# Autodesk Inventor assembly: robot
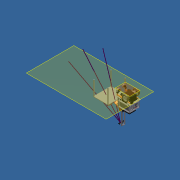
[picture p0: Inventor's stored thumbnail of the model, 180x180]
Saved by Autodesk Inventor 2012 (Build 160160000, 160)
## iProperties
Created: 2012-03-08
Part Number: robot
Document SubType Name: Assembly
Designer: esv
Mass: 187059 g
Surface Area: 125343 cm^2
Volume: 160092 cm^3
Density: 1.16845 g/cm^3
Author: esv
## Documents named in this file (22)
- C:\Users\Ed\Documents\masters\CAD\robot.iam
- C:\Users\Ed\Documents\masters\CAD\Frame\frame bracket.ipt
- C:\Users\Ed\Documents\masters\CAD\Invacare\invacare assy.iam
- C:\Users\Ed\Documents\masters\CAD\IRC5\IRC5_Compact.ipt
- C:\Users\Ed\Documents\masters\CAD\PC\PC.ipt
- C:\Users\Ed\Documents\masters\CAD\SICK\SICK LMS291.ipt
- C:\Users\Ed\Documents\masters\CAD\IRB120\IRB120.iam
- C:\Users\Ed\Documents\masters\CAD\Frame\back frame plate.ipt
- C:\Users\Ed\Documents\masters\CAD\Frame\front frame plate.ipt
- C:\Users\Ed\Documents\masters\CAD\Frame\top plate.ipt
- C:\Users\Ed\Documents\masters\CAD\Pneumatics\compressor\compressor.iam
- C:\Users\Ed\Documents\masters\CAD\Spike\Spike H.iam
- C:\Users\Ed\Documents\masters\CAD\Breaker\Breaker.iam
- C:\Users\Ed\Documents\masters\CAD\Router\router keepout.ipt
- C:\Users\Ed\Documents\masters\CAD\Frame\short frame bracket.ipt
- C:\Users\Ed\Documents\masters\CAD\base plate.iam
- C:\Users\Ed\Documents\masters\CAD\Gripper\gripper.iam
- C:\Users\Ed\Documents\masters\CAD\al_frame.iam
- C:\Users\Ed\Documents\masters\CAD\Gripper\gripper jaw.iam
- C:\Users\Ed\Documents\masters\CAD\Kinect\acrylic kinect bracket.iam
- C:\Users\Ed\Documents\masters\CAD\Kinect\Kinect.ipt
- C:\Users\Ed\Documents\masters\CAD\objects\table.ipt
## Components (26 placed, 21 different names)
1. frame bracket:1 — Flush:5, Mate:72, Flush:56, Mate:74, Mate:132
2. frame bracket:4 — Flush:5, Flush:57, Mate:75, Mate:76
3. invacare assy:1 [sub-assembly] — Flush:96, Tangent:8, Mate:97, Mate:143, Mate:144, Mate:145
4. IRC5_Compact:1 — Flush:2, Mate:122, Mate:126
5. PC:1 — Mate:36, Flush:63, Flush:91
6. SICK LMS291:1 — Mate:118, Insert:12
7. IRB120:1 [sub-assembly] — Insert:10, Insert:11, Mate:120, Tangent:7, Flush:145
8. back frame plate:1 — Flush:82, Insert:7, Flush:88, Flush:89, Flush:96, Tangent:8, Flush:98
9. back frame plate:2 — Insert:6, Flush:87, Flush:88, Flush:90, Flush:100
10. front frame plate:1 — Flush:57, Mate:75, Mate:76, Flush:89, Mate:97, Flush:98, Flush:99
11. front frame plate:2 — Mate:72, Flush:56, Mate:74, Flush:90, Flush:99, Flush:100
12. top plate:1 — Mate:36, Mate:80, Flush:63, Mate:81, Insert:1, Insert:2, Insert:3, Mate:82, Insert:4, Insert:5, Flush:64, Mate:121, Flush:85, Flush:86, Flush:91
13. compressor:1 [sub-assembly] — Mate:80, Insert:2, Insert:3
14. Spike H:1 [sub-assembly] — Mate:81, Insert:1
15. Breaker:1 [sub-assembly] — Mate:82, Insert:4, Insert:5
16. router keepout:1 — Flush:64, Mate:83, Mate:119
17. short frame bracket:1 — Insert:6, Flush:87, Mate:127, Mate:129, Mate:130
18. short frame bracket:2 — Flush:82, Insert:7, Mate:131
19. base plate:1 [sub-assembly] — Mate:123, Mate:124, Mate:125, Mate:126
20. gripper:2 [sub-assembly] — Insert:10, Insert:11, Mate:135, Flush:94, Flush:95
21. al_frame:1 [sub-assembly] — Mate:119, Mate:120, Tangent:7, Mate:121, Flush:85, Flush:86, Mate:122, Insert:12, Mate:123, Mate:124, Mate:125, Mate:127, Mate:129, Mate:130, Mate:131, Mate:132, Mate:137, Mate:138, Flush:101, Mate:146, Flush:146
22. gripper jaw:1 [sub-assembly] — Flush:92, Flush:93, Mate:135, Flush:94, Mate:136
23. gripper jaw:2 [sub-assembly] — Flush:92, Flush:93, Mate:136, Flush:95, Mate:147
24. acrylic kinect bracket:1 [sub-assembly] — Mate:137, Mate:138, Flush:101, Insert:13, Insert:14
25. Kinect:1 — Insert:13, Insert:14
26. table:1 — Mate:145, Mate:146, Flush:146, Mate:147
## Relationships (73: Mate 34, Flush 25, Insert 12, Tangent 2)
- Flush:2 (-225 mm): IRC5_Compact:1
- Flush:5: frame bracket:1 ↔ frame bracket:4
- Mate:36: PC:1 ↔ top plate:1
- Mate:72: frame bracket:1 ↔ front frame plate:2
- Flush:56: frame bracket:1 ↔ front frame plate:2
- Mate:74: frame bracket:1 ↔ front frame plate:2
- Flush:57: frame bracket:4 ↔ front frame plate:1
- Mate:75: frame bracket:4 ↔ front frame plate:1
- Mate:76: frame bracket:4 ↔ front frame plate:1
- Mate:80: top plate:1 ↔ compressor:1
- Flush:63 (-50.8 mm): PC:1 ↔ top plate:1
- Mate:81: top plate:1 ↔ Spike H:1
- Insert:1: top plate:1 ↔ Spike H:1
- Insert:2: top plate:1 ↔ compressor:1
- Insert:3: top plate:1 ↔ compressor:1
- Mate:82: top plate:1 ↔ Breaker:1
- Insert:4: top plate:1 ↔ Breaker:1
- Insert:5: top plate:1 ↔ Breaker:1
- Flush:64 (-304.8 mm): top plate:1 ↔ router keepout:1
- Mate:83: router keepout:1
- Insert:6: back frame plate:2 ↔ short frame bracket:1
- Flush:82: back frame plate:1 ↔ short frame bracket:2
- Insert:7: back frame plate:1 ↔ short frame bracket:2
- Mate:118: SICK LMS291:1
- Insert:10: IRB120:1 ↔ gripper:2
- Insert:11: IRB120:1 ↔ gripper:2
- Mate:119: router keepout:1 ↔ al_frame:1
- Mate:120: IRB120:1 ↔ al_frame:1
- Tangent:7: IRB120:1 ↔ al_frame:1
- Mate:121: top plate:1 ↔ al_frame:1
- Flush:85: top plate:1 ↔ al_frame:1
- Flush:86: top plate:1 ↔ al_frame:1
- Mate:122: IRC5_Compact:1 ↔ al_frame:1
- Insert:12: SICK LMS291:1 ↔ al_frame:1
- Mate:123: base plate:1 ↔ al_frame:1
- Mate:124: base plate:1 ↔ al_frame:1
- Mate:125: base plate:1 ↔ al_frame:1
- Mate:126: IRC5_Compact:1 ↔ base plate:1
- Flush:87: back frame plate:2 ↔ short frame bracket:1
- Flush:88: back frame plate:1 ↔ back frame plate:2
- Flush:89: back frame plate:1 ↔ front frame plate:1
- Flush:90: back frame plate:2 ↔ front frame plate:2
- Mate:127: short frame bracket:1 ↔ al_frame:1
- Mate:129: short frame bracket:1 ↔ al_frame:1
- Mate:130: short frame bracket:1 ↔ al_frame:1
- Mate:131: short frame bracket:2 ↔ al_frame:1
- Flush:91 (50.8 mm): PC:1 ↔ top plate:1
- Mate:132: frame bracket:1 ↔ al_frame:1
- Flush:92: gripper jaw:1 ↔ gripper jaw:2
- Flush:93: gripper jaw:1 ↔ gripper jaw:2
- Mate:135: gripper:2 ↔ gripper jaw:1
- Flush:94: gripper:2 ↔ gripper jaw:1
- Mate:136 (63.5 mm): gripper jaw:1 ↔ gripper jaw:2
- Flush:95: gripper:2 ↔ gripper jaw:2
- Flush:96 (88.9 mm): invacare assy:1 ↔ back frame plate:1
- Tangent:8: invacare assy:1 ↔ back frame plate:1
- Mate:97: invacare assy:1 ↔ front frame plate:1
- Flush:98: back frame plate:1 ↔ front frame plate:1
- Flush:99: front frame plate:1 ↔ front frame plate:2
- Flush:100: back frame plate:2 ↔ front frame plate:2
- Mate:137: al_frame:1 ↔ acrylic kinect bracket:1
- Mate:138: al_frame:1 ↔ acrylic kinect bracket:1
- Flush:101 (3.175 mm): al_frame:1 ↔ acrylic kinect bracket:1
- Mate:142
- Mate:143 (-317.5 mm): invacare assy:1
- Mate:144: invacare assy:1
- Flush:145 (812.8 mm): IRB120:1
- Mate:145: invacare assy:1 ↔ table:1
- Mate:146 (304.8 mm): al_frame:1 ↔ table:1
- Flush:146 (-203.2 mm): al_frame:1 ↔ table:1
- Mate:147 (25.4 mm): gripper jaw:2 ↔ table:1
- Insert:13: acrylic kinect bracket:1 ↔ Kinect:1
- Insert:14: acrylic kinect bracket:1 ↔ Kinect:1
